# Autodesk Inventor assembly: OUTK_000_Assembly
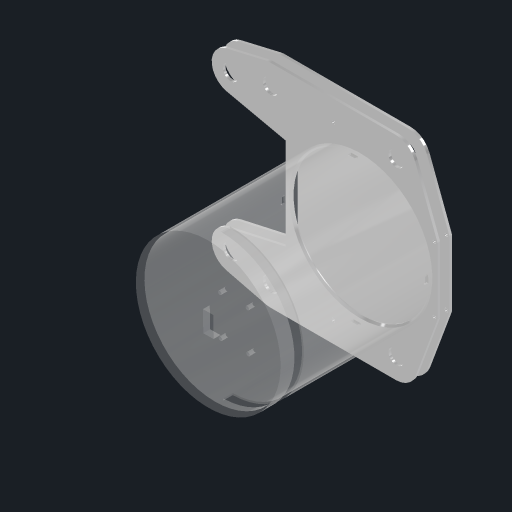
[picture p0: Inventor's stored thumbnail of the model, 512x512]
Saved by Autodesk Inventor 2024.2 (Build 282272000, 272)
## iProperties
Created: 2024-11-24
Part Number: OUTK_000_Assembly
Document SubType Name: Assembly
Designer: Bryan
Mass: 4116.39 g
Surface Area: 9620.73 cm^2
Volume: 2289.12 cm^3
Density: 1.79824 g/cm^3
Author: Bryan
## Documents named in this file (4)
- C:\Users\bobsb\OneDrive\Documents\GitHub\1622-2024-Casino-Clash-CAD-A-Thon\Outtake\OUTK_000_Assembly.iam
- C:\Users\bobsb\OneDrive\Documents\GitHub\1622-2024-Casino-Clash-CAD-A-Thon\Outtake\OUTK_002_ShotPlateNoReceptacle.ipt
- C:\Users\bobsb\OneDrive\Documents\GitHub\1622-2024-Casino-Clash-CAD-A-Thon\Outtake\OUTK_002_ShotPlateReceptacle.ipt
- C:\Users\bobsb\OneDrive\Documents\GitHub\1622-2024-Casino-Clash-CAD-A-Thon\Outtake\OUTK_001_ChipBucket.ipt
## Components (3 placed, 3 different names)
1. OUTK_002_ShotPlateNoReceptacle:1 — Mate:1, Mate:2, Mate:5
2. OUTK_002_ShotPlateReceptacle:1 — Mate:1, Mate:2, Mate:3, Mate:4, Mate:5
3. OUTK_001_ChipBucket:1 — Mate:3, Mate:4
## Relationships (5: Mate 5)
- Mate:1: OUTK_002_ShotPlateNoReceptacle:1 ↔ OUTK_002_ShotPlateReceptacle:1
- Mate:2: OUTK_002_ShotPlateNoReceptacle:1 ↔ OUTK_002_ShotPlateReceptacle:1
- Mate:3: OUTK_002_ShotPlateReceptacle:1 ↔ OUTK_001_ChipBucket:1
- Mate:4: OUTK_002_ShotPlateReceptacle:1 ↔ OUTK_001_ChipBucket:1
- Mate:5 (17.145 mm): OUTK_002_ShotPlateNoReceptacle:1 ↔ OUTK_002_ShotPlateReceptacle:1
